# Autodesk Inventor assembly: sp16-2p connector male
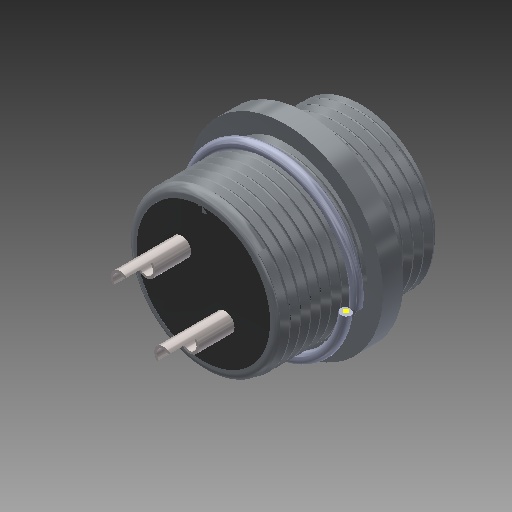
[picture p0: Inventor's stored thumbnail of the model, 512x512]
Saved by Autodesk Inventor 2018 (Build 220112000, 112)
## iProperties
Created: 2019-04-03
Part Number: sp16-2p connector male
Document SubType Name: Assembly
Designer: ZEUSLAP
Author: ZEUSLAP
## Documents named in this file (4)
- C:\Users\ZEUSLAP\YandexDisk\Inventor\solar_harvester_145x145\parts\sp16 waterproof connector\sp16-2p connector male.iam
- C:\Users\ZEUSLAP\YandexDisk\Inventor\solar_harvester_145x145\parts\sp16 waterproof connector\parts\2 pin body male.ipt
- C:\Users\ZEUSLAP\YandexDisk\Inventor\solar_harvester_145x145\parts\sp16 waterproof connector\parts\male_connector_body_metal.ipt
- C:\Users\ZEUSLAP\YandexDisk\Inventor\solar_harvester_145x145\parts\sp16 waterproof connector\parts\male_connector_spring_washer.ipt
## Components (3 placed, 3 different names)
1. 2 pin body male:1 — Rotational:1
2. male_connector_body_metal:1 — Rotational:1, Mate:2
3. male_connector_spring_washer:1 — Mate:2
## Relationships (2: RevoluteJoint 1, Mate 1)
- Rotational:1 [RevoluteJoint]: 2 pin body male:1 ↔ male_connector_body_metal:1
- Mate:2: male_connector_body_metal:1 ↔ male_connector_spring_washer:1
